# Autodesk Inventor assembly: CT2X2
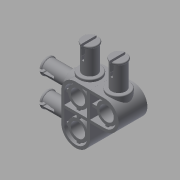
[picture p0: Inventor's stored thumbnail of the model, 180x180]
Saved by Autodesk Inventor 2019.3 (Build 233278000, 278)
## iProperties
Created: 2019-01-31
Part Number: CT2X2
Document SubType Name: Assembly
Designer: Varga Daniel
Author: Varga Daniel
Vertical_hole_count: 3,000 ul
Horizontal_hole_count: 3,000 ul
## Documents named in this file (8)
- C:\!_Dani\!_cloud\OneDrive\!_munka\Revolution\RevvyDemoKit\Structural parts\Connector Boxes\Connector triangle\CT2+x2+\CT2x2.iam
- C:\!_Dani\!_cloud\OneDrive\!_munka\Revolution\RevvyDemoKit\Structural parts\Beams\beam_single_end_part.ipt
- C:\!_Dani\!_cloud\OneDrive\!_munka\Revolution\RevvyDemoKit\Structural parts\Connetor Pins\Connector_pin_stick.ipt
- C:\!_Dani\!_cloud\OneDrive\!_munka\Revolution\RevvyDemoKit\Structural parts\Connector Boxes\Connector_box_collar\Connector_box_collar-one_side.ipt
- C:\!_Dani\!_cloud\OneDrive\!_munka\Revolution\RevvyDemoKit\Structural parts\Connector Boxes\Connector_box_collar.ipt
- C:\!_Dani\!_cloud\OneDrive\!_munka\Revolution\RevvyDemoKit\Structural parts\Connector Boxes\Connector triangle\Connector_triangle_L_base.ipt
- C:\!_Dani\!_cloud\OneDrive\!_munka\Revolution\RevvyDemoKit\Structural parts\Connector Boxes\Connector_box_collar\Connector_box_collar-None.ipt
- C:\!_Dani\!_cloud\OneDrive\!_munka\Revolution\RevvyDemoKit\Structural parts\Connector Boxes\Connector triangle\CT2+x2+.iam
## Components (13 placed, 5 different names)
1. Connector_triangle_L_base:1 — Mate:40, Mate:41, Angle:5, Mate:42, Mate:43, Angle:6, Flush:3, Flush:4, Mate:49, Flush:7, Flush:8, Mate:55
2. beam_single_end_part:1 — Mate:37, Mate:38, Mate:39, Angle:4, Flush:7, Flush:8, Mate:55
3. beam_single_end_part:2 — Mate:28, Mate:29, Angle:1, Mate:36, Flush:3, Flush:4, Mate:49
4. Connector_box_collar-one_side:1 — Mate:18, Mate:19, Mate:37, Mate:38
5. Connector_pin_stick:2 — Mate:18, Mate:19, Mate:39, Angle:4
6. Connector_box_collar-one_side:3 — Mate:41
7. Connector_pin_stick:3 — Mate:40, Angle:5
8. Connector_box_collar-one_side:4 — Mate:43
9. Connector_pin_stick:4 — Mate:42, Angle:6
10. Connector_box_collar-one_side:5 — Mate:28, Mate:29
11. Connector_pin_stick:5 — Angle:1, Mate:36
12. Connector_box_collar-None:6
13. Connector_box_collar-None:7
## Relationships (28: Mate 20, Angle 4, Flush 4)
- Mate:18: Connector_box_collar-one_side:1 ↔ Connector_pin_stick:2
- Mate:19: Connector_box_collar-one_side:1 ↔ Connector_pin_stick:2
- [Mate]: Connector_box_collar-one_side:3 ↔ Connector_pin_stick:3
- [Mate]: Connector_box_collar-one_side:3 ↔ Connector_pin_stick:3
- [Mate]: Connector_box_collar-one_side:4 ↔ Connector_pin_stick:4
- [Mate]: Connector_box_collar-one_side:4 ↔ Connector_pin_stick:4
- [Mate]: Connector_box_collar-one_side:5 ↔ Connector_pin_stick:5
- [Mate]: Connector_box_collar-one_side:5 ↔ Connector_pin_stick:5
- Mate:28: beam_single_end_part:2 ↔ Connector_box_collar-one_side:5
- Mate:29: beam_single_end_part:2 ↔ Connector_box_collar-one_side:5
- Angle:1 (0 deg): beam_single_end_part:2 ↔ Connector_pin_stick:5
- Mate:36: beam_single_end_part:2 ↔ Connector_pin_stick:5
- Mate:37: beam_single_end_part:1 ↔ Connector_box_collar-one_side:1
- Mate:38: beam_single_end_part:1 ↔ Connector_box_collar-one_side:1
- Mate:39: beam_single_end_part:1 ↔ Connector_pin_stick:2
- Angle:4 (0 deg): beam_single_end_part:1 ↔ Connector_pin_stick:2
- Mate:40: Connector_triangle_L_base:1 ↔ Connector_pin_stick:3
- Mate:41: Connector_triangle_L_base:1 ↔ Connector_box_collar-one_side:3
- Angle:5 (0 deg): Connector_triangle_L_base:1 ↔ Connector_pin_stick:3
- Mate:42: Connector_triangle_L_base:1 ↔ Connector_pin_stick:4
- Mate:43: Connector_triangle_L_base:1 ↔ Connector_box_collar-one_side:4
- Angle:6 (0 deg): Connector_triangle_L_base:1 ↔ Connector_pin_stick:4
- Flush:3: Connector_triangle_L_base:1 ↔ beam_single_end_part:2
- Flush:4: Connector_triangle_L_base:1 ↔ beam_single_end_part:2
- Mate:49: Connector_triangle_L_base:1 ↔ beam_single_end_part:2
- Flush:7: Connector_triangle_L_base:1 ↔ beam_single_end_part:1
- Flush:8: Connector_triangle_L_base:1 ↔ beam_single_end_part:1
- Mate:55: Connector_triangle_L_base:1 ↔ beam_single_end_part:1
## Named parameters: Vertical_hole_count = 3, Horizontal_hole_count = 3, d53_d49 = 0 mm, d54_d50 = 0 mm, d55_d49 = 0 mm, d56_d50 = 0 mm, d57_d49 = 0 mm, d58_d50 = 0 mm
